# Autodesk Inventor assembly: Assembly2
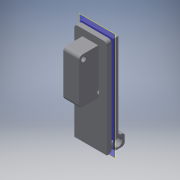
[picture p0: Inventor's stored thumbnail of the model, 180x180]
Saved by Autodesk Inventor 2019 (Build 230136000, 136)
## iProperties
Created: 2021-01-21
Part Number: Assembly2
Material: Genérico
Document SubType Name: Assembly
Designer: Juan M. Casillas
Author: Juan M. Casillas
## Documents named in this file (4)
- K:\3DPrinting\3DModels\shifter\Assembly2.iam
- K:\3DPrinting\3DModels\shifter\plate1.ipt
- K:\3DPrinting\3DModels\shifter\lever.ipt
- K:\3DPrinting\3DModels\shifter\microswitch.ipt
## Components (3 placed, 3 different names)
1. plate1:1 — Flush:1, Mate:1, Mate:2, Mate:3
2. lever:1 — Flush:2, Flush:3
3. microswitch:1 — Mate:1, Mate:2, Mate:3
## Relationships (6: Flush 3, Mate 3)
- Flush:1 (1 mm): plate1:1
- Flush:2: lever:1
- Flush:3: lever:1
- Mate:1: plate1:1 ↔ microswitch:1
- Mate:2: plate1:1 ↔ microswitch:1
- Mate:3 (-1 mm): plate1:1 ↔ microswitch:1
